# Autodesk Inventor assembly: mid_brace
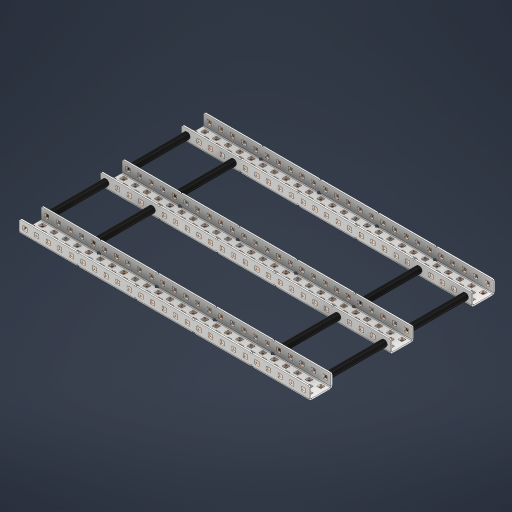
[picture p0: Inventor's stored thumbnail of the model, 512x512]
Saved by Autodesk Inventor 2024 (Build 280153000, 153)
## iProperties
Created: 2023-10-18
Part Number: mid_brace
Document SubType Name: Assembly
Designer: Averey Ku
Author: Averey Ku
## Documents named in this file (4)
- D:\vex_robotics\hardware\cad\goated_v0.1\chassis\mid_brace.iam
- D:\vex_robotics\hardware\cad\VEX-CAD-Inventor-1.41\Structure\Standoff\Standoff 2.50.ipt
- D:\vex_robotics\hardware\cad\VEX-CAD-Inventor-1.41\Structure\Standoff.ipt
- D:\vex_robotics\hardware\cad\VEX-CAD-Inventor-1.41\Structure\C Channel\Aluminum 1x2x1\Alu C 1x2x1x25.ipt
## Components (11 placed, 2 different names)
1. Standoff 2.50:1 — Insert:1, Insert:3
2. Standoff 2.50:2 — Insert:5
3. Standoff 2.50:3 — Insert:4
4. Standoff 2.50:4 — Insert:2, Mate:1
5. Standoff 2.50:5 — Insert:6, Insert:10
6. Standoff 2.50:6 — Insert:7, Mate:2
7. Standoff 2.50:7 — Insert:8
8. Standoff 2.50:8 — Insert:9
9. Alu C 1x2x1x25:1 — Insert:1, Insert:2, Insert:4, Insert:5
10. Alu C 1x2x1x25:2 — Insert:3, Mate:1, Insert:6, Insert:7, Insert:8, Insert:9
11. Alu C 1x2x1x25:3 — Insert:10, Mate:2
## Relationships (12: Insert 10, Mate 2)
- Insert:1: Standoff 2.50:1 ↔ Alu C 1x2x1x25:1
- Insert:2: Standoff 2.50:4 ↔ Alu C 1x2x1x25:1
- Insert:3: Standoff 2.50:1 ↔ Alu C 1x2x1x25:2
- Mate:1: Standoff 2.50:4 ↔ Alu C 1x2x1x25:2
- Insert:4: Standoff 2.50:3 ↔ Alu C 1x2x1x25:1
- Insert:5: Standoff 2.50:2 ↔ Alu C 1x2x1x25:1
- Insert:6: Standoff 2.50:5 ↔ Alu C 1x2x1x25:2
- Insert:7: Standoff 2.50:6 ↔ Alu C 1x2x1x25:2
- Insert:8: Standoff 2.50:7 ↔ Alu C 1x2x1x25:2
- Insert:9: Standoff 2.50:8 ↔ Alu C 1x2x1x25:2
- Insert:10: Standoff 2.50:5 ↔ Alu C 1x2x1x25:3
- Mate:2: Standoff 2.50:6 ↔ Alu C 1x2x1x25:3
